# Autodesk Inventor assembly: rob_base
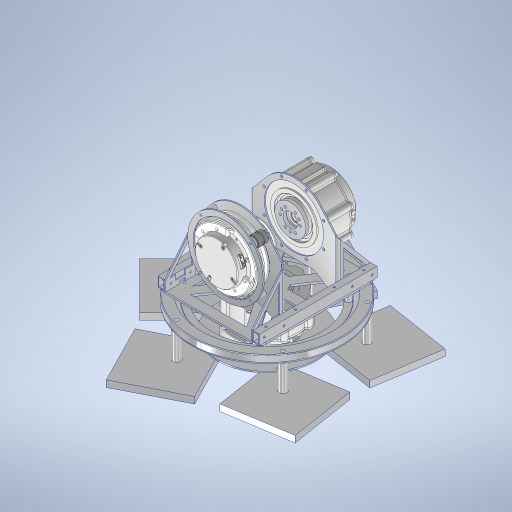
[picture p0: Inventor's stored thumbnail of the model, 512x512]
Saved by Autodesk Inventor 2024 (Build 280153000, 153)
## iProperties
Created: 2025-01-31
Part Number: rob_base
Document SubType Name: Assembly
Designer: tanoue_kota
Mass: 2971.99 g
Surface Area: 4971.73 cm^2
Volume: 574.145 cm^3
Density: 5.17638 g/cm^3
Author: tanoue_kota
## Documents named in this file (22)
- C:\Users\田之上巧太\Documents\Inventor\RobArm\rob_base\rob_base.iam
- C:\Users\田之上巧太\Documents\Inventor\RobArm\rob_base\rob_base_parameter.ipt
- C:\Users\田之上巧太\Documents\Inventor\RobArm\Actuator\RS03\RS03.iam
- C:\Users\田之上巧太\Documents\Inventor\RobArm\rob_base\base_plate1.ipt
- C:\Users\田之上巧太\Documents\Inventor\RobArm\rob_base\base_plate2.ipt
- C:\Users\田之上巧太\Documents\Inventor\RobArm\rob_base\base_plate3.ipt
- C:\Users\田之上巧太\Documents\Inventor\RobArm\rob_base\base_part1.ipt
- C:\Users\田之上巧太\Documents\Inventor\RobArm\rob_base\base_part2.ipt
- C:\Users\田之上巧太\Documents\Inventor\RobArm\rob_base\base_plate4.ipt
- C:\Users\田之上巧太\Documents\Inventor\RobArm\rob_base\base_pipe1.ipt
- C:\Users\田之上巧太\Documents\Inventor\RobArm\Actuator\RS02\RS02.iam
- C:\Users\田之上巧太\Documents\Inventor\RobArm\BasicParts\TurnTable\hf23sp_0\hf23sp_0.iam
- C:\Users\田之上巧太\Documents\Inventor\RobArm\rob_base\base_plate5.ipt
- C:\Users\田之上巧太\Documents\Inventor\RobArm\rob_base\base_part3.ipt
- C:\Users\田之上巧太\Documents\Inventor\RobArm\rob_base\base_part4.ipt
- C:\Users\田之上巧太\Documents\Inventor\RobArm\rob_base\base_part5.ipt
- C:\Users\田之上巧太\Documents\Inventor\RobArm\rob_base\base_part6.ipt
- C:\Users\田之上巧太\Documents\Inventor\RobArm\rob_base\base_part7.ipt
- C:\Users\田之上巧太\Documents\Inventor\RobArm\rob_base\Bearing_small.ipt
- C:\Users\田之上巧太\Documents\Inventor\RobArm\rob_base\base_plate6.ipt
- C:\Users\田之上巧太\Documents\Inventor\RobArm\rob_base\base_part8.ipt
- C:\Users\田之上巧太\Documents\Inventor\RobArm\rob_base\base_plate7.ipt
## Components (39 placed, 21 different names)
1. rob_base_parameter:1
2. RS03:1 [sub-assembly] — 回転:1, 回転:2, 回転:3, 回転:4
3. base_plate1:1 — 回転:1, 回転:2, フラッシュ:1, フラッシュ:2, 回転:15, 回転:16
4. base_plate2:1 — 回転:3, 回転:4, メイト:2, メイト:13, メイト:1
5. base_plate3:1 — 回転:5, 回転:6, 回転:7, 回転:8, フラッシュ:1, フラッシュ:2, 回転:17, フラッシュ:4, 回転:22, メイト:7
6. base_part1:1 — 回転:5, 回転:12, メイト:3, メイト:6, メイト:8, メイト:9, メイト:11
7. base_part1:2 — 回転:8
8. base_part1:3 — 回転:7, 回転:11
9. base_part1:4 — 回転:6
10. base_part2:1 — 回転:18, 回転:19, フラッシュ:5
11. base_plate4:1 — 回転:11, 回転:12, フラッシュ:5, メイト:4
12. base_pipe1:1 — 回転:15, 回転:22, 回転:28
13. base_pipe1:2 — 回転:16, 回転:17, フラッシュ:4, 回転:21
14. RS02:1 [sub-assembly] — 回転:18, 回転:19, メイト:2, 回転:30, 回転:31, メイト:13
15. hf23sp_0:2 [sub-assembly] — 回転:23, 回転:24, 回転:25, 回転:26, 回転:34, 回転:35, 回転:37, 回転:38, メイト:14
16. base_plate5:1 — 回転:21, 回転:27, 回転:28, 回転:29, 回転:41, 回転:42
17. base_part3:1 — 回転:23
18. base_part3:2 — 回転:24, 回転:27
19. base_part3:3 — 回転:26
20. base_part3:4 — 回転:25, 回転:29
21. base_part4:1 — 回転:30, 回転:31, メイト:1
22. RS03:2 [sub-assembly] — 回転:41, 回転:42, 回転:43, 回転:44
23. base_part5:1 — 回転:34, 回転:40
24. base_part5:2 — 回転:35, フラッシュ:6, 回転:54
25. base_part5:3 — フラッシュ:6, 回転:49, メイト:14
26. base_part5:4 — 回転:37, 回転:51
27. base_part5:5 — 回転:38, 回転:52
28. base_part6:1 — メイト:3, メイト:4, メイト:5, メイト:10
29. base_part7:1 — メイト:5, メイト:6, メイト:12
30. base_part6:2 — メイト:7, メイト:8
31. Bearing_small:1 — メイト:9, メイト:10
32. Bearing_small:2 — メイト:11, メイト:12
33. base_plate6:1 — 回転:40, 回転:47
34. base_part8:1 — 回転:43, 回転:44, 回転:45, 回転:46
35. base_plate7:1 — 回転:45, 回転:46, 回転:47, 回転:48, 回転:50, 回転:53, 回転:55
36. base_plate6:2 — 回転:48, 回転:49
37. base_plate6:3 — 回転:50, 回転:51
38. base_plate6:4 — 回転:52, 回転:53
39. base_plate6:5 — 回転:54, 回転:55
## Relationships (65: RevoluteJoint 46, Mate 14, Flush 5)
- 回転:1 [RevoluteJoint]: RS03:1 ↔ base_plate1:1
- 回転:2 [RevoluteJoint]: RS03:1 ↔ base_plate1:1
- 回転:3 [RevoluteJoint]: RS03:1 ↔ base_plate2:1
- 回転:4 [RevoluteJoint]: RS03:1 ↔ base_plate2:1
- 回転:5 [RevoluteJoint]: base_plate3:1 ↔ base_part1:1
- 回転:6 [RevoluteJoint]: base_plate3:1 ↔ base_part1:4
- 回転:7 [RevoluteJoint]: base_plate3:1 ↔ base_part1:3
- 回転:8 [RevoluteJoint]: base_plate3:1 ↔ base_part1:2
- フラッシュ:1 [Flush]: base_plate1:1 ↔ base_plate3:1
- フラッシュ:2 [Flush]: base_plate1:1 ↔ base_plate3:1
- 回転:11 [RevoluteJoint]: base_part1:3 ↔ base_plate4:1
- 回転:12 [RevoluteJoint]: base_part1:1 ↔ base_plate4:1
- 回転:15 [RevoluteJoint]: base_plate1:1 ↔ base_pipe1:1
- 回転:16 [RevoluteJoint]: base_plate1:1 ↔ base_pipe1:2
- 回転:17 [RevoluteJoint]: base_plate3:1 ↔ base_pipe1:2
- フラッシュ:4 [Flush]: base_plate3:1 ↔ base_pipe1:2
- 回転:18 [RevoluteJoint]: base_part2:1 ↔ RS02:1
- 回転:19 [RevoluteJoint]: base_part2:1 ↔ RS02:1
- メイト:1 [Mate]: base_plate2:1 ↔ base_part4:1
- メイト:2 [Mate] (71 mm): base_plate2:1 ↔ RS02:1
- 回転:21 [RevoluteJoint]: base_pipe1:2 ↔ base_plate5:1
- 回転:22 [RevoluteJoint]: base_plate3:1 ↔ base_pipe1:1
- 回転:23 [RevoluteJoint]: hf23sp_0:2 ↔ base_part3:1
- 回転:24 [RevoluteJoint]: hf23sp_0:2 ↔ base_part3:2
- 回転:25 [RevoluteJoint]: hf23sp_0:2 ↔ base_part3:4
- 回転:26 [RevoluteJoint]: hf23sp_0:2 ↔ base_part3:3
- 回転:27 [RevoluteJoint]: base_plate5:1 ↔ base_part3:2
- 回転:28 [RevoluteJoint]: base_pipe1:1 ↔ base_plate5:1
- 回転:29 [RevoluteJoint]: base_plate5:1 ↔ base_part3:4
- 回転:30 [RevoluteJoint]: RS02:1 ↔ base_part4:1
- 回転:31 [RevoluteJoint]: RS02:1 ↔ base_part4:1
- 回転:34 [RevoluteJoint]: hf23sp_0:2 ↔ base_part5:1
- 回転:35 [RevoluteJoint]: hf23sp_0:2 ↔ base_part5:2
- 回転:37 [RevoluteJoint]: hf23sp_0:2 ↔ base_part5:4
- 回転:38 [RevoluteJoint]: hf23sp_0:2 ↔ base_part5:5
- フラッシュ:5 [Flush] (-2.5 mm): base_part2:1 ↔ base_plate4:1
- メイト:3 [Mate]: base_part1:1 ↔ base_part6:1
- メイト:4 [Mate]: base_plate4:1 ↔ base_part6:1
- メイト:5 [Mate] (6 mm): base_part6:1 ↔ base_part7:1
- メイト:6 [Mate]: base_part1:1 ↔ base_part7:1
- メイト:7 [Mate]: base_plate3:1 ↔ base_part6:2
- メイト:8 [Mate]: base_part1:1 ↔ base_part6:2
- メイト:9 [Mate]: base_part1:1 ↔ Bearing_small:1
- メイト:10 [Mate]: base_part6:1 ↔ Bearing_small:1
- メイト:11 [Mate]: base_part1:1 ↔ Bearing_small:2
- メイト:12 [Mate]: base_part7:1 ↔ Bearing_small:2
- メイト:13 [Mate] (71 mm): base_plate2:1 ↔ RS02:1
- 回転:40 [RevoluteJoint]: base_part5:1 ↔ base_plate6:1
- 回転:41 [RevoluteJoint]: base_plate5:1 ↔ RS03:2
- 回転:42 [RevoluteJoint]: base_plate5:1 ↔ RS03:2
- 回転:43 [RevoluteJoint]: RS03:2 ↔ base_part8:1
- 回転:44 [RevoluteJoint]: RS03:2 ↔ base_part8:1
- 回転:45 [RevoluteJoint]: base_part8:1 ↔ base_plate7:1
- 回転:46 [RevoluteJoint]: base_part8:1 ↔ base_plate7:1
- 回転:47 [RevoluteJoint]: base_plate6:1 ↔ base_plate7:1
- 回転:48 [RevoluteJoint]: base_plate7:1 ↔ base_plate6:2
- フラッシュ:6 [Flush]: base_part5:2 ↔ base_part5:3
- 回転:49 [RevoluteJoint]: base_part5:3 ↔ base_plate6:2
- メイト:14 [Mate]: hf23sp_0:2 ↔ base_part5:3
- 回転:50 [RevoluteJoint]: base_plate7:1 ↔ base_plate6:3
- 回転:51 [RevoluteJoint]: base_part5:4 ↔ base_plate6:3
- 回転:52 [RevoluteJoint]: base_part5:5 ↔ base_plate6:4
- 回転:53 [RevoluteJoint]: base_plate7:1 ↔ base_plate6:4
- 回転:54 [RevoluteJoint]: base_part5:2 ↔ base_plate6:5
- 回転:55 [RevoluteJoint]: base_plate7:1 ↔ base_plate6:5
